# Autodesk Inventor assembly: linkage_system_test
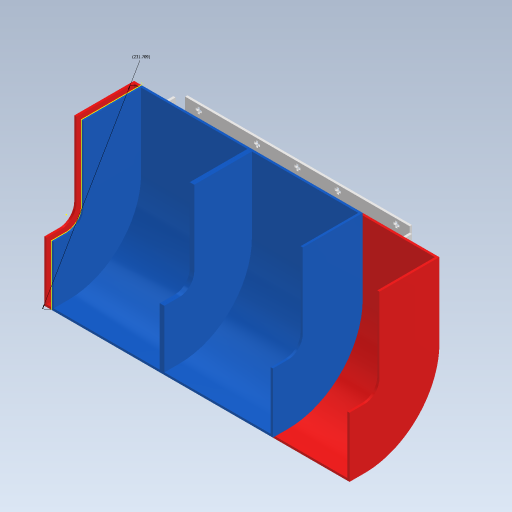
[picture p0: Inventor's stored thumbnail of the model, 512x512]
Saved by Autodesk Inventor 2023 (Build 270158000, 158)
## iProperties
Created: 2023-05-05
Part Number: linkage_system_test
Document SubType Name: Assembly
Designer: 陳詩穎
Author: 陳詩穎
## Documents named in this file (14)
- C:\Users\Johnny Jou\Documents\GitHub\Areo_Rider_Cabin\Expansion\test\linkage_system_test.iam
- C:\Users\Johnny Jou\Documents\GitHub\Areo_Rider_Cabin\Expansion\test\plate_expansion.ipt
- C:\Users\Johnny Jou\Documents\GitHub\Areo_Rider_Cabin\Expansion\test\零件1.ipt
- C:\Users\Johnny Jou\Documents\GitHub\Areo_Rider_Cabin\Expansion\test\adjustable.ipt
- C:\Users\Johnny Jou\Documents\GitHub\Areo_Rider_Cabin\Expansion\test\零件4.ipt
- C:\Users\Johnny Jou\Documents\GitHub\Areo_Rider_Cabin\Expansion\test\零件5.ipt
- C:\Users\Johnny Jou\Documents\GitHub\Areo_Rider_Cabin\Expansion\test\零件7.ipt
- C:\Users\Johnny Jou\Documents\GitHub\Areo_Rider_Cabin\Airfoil & Nuzzle\nuzzle\nuzzle_v2_0327.ipt
- C:\Users\Johnny Jou\Documents\GitHub\Areo_Rider_Cabin\Airfoil & Nuzzle\nuzzle\nuzzle_v2_0516.ipt
- C:\Users\Johnny Jou\Documents\GitHub\Areo_Rider_Cabin\Airfoil & Nuzzle\nuzzle\nuzzle_v2_0516_2.ipt
- C:\Users\Johnny Jou\Documents\GitHub\Areo_Rider_Cabin\Expansion\test\零件8.ipt
- C:\Users\Johnny Jou\Documents\GitHub\Areo_Rider_Cabin\Expansion\test\零件9.ipt
- C:\Users\Johnny Jou\Documents\GitHub\Areo_Rider_Cabin\Expansion\test\零件10.ipt
- C:\Users\Johnny Jou\Documents\GitHub\Areo_Rider_Cabin\Expansion\test\零件12.ipt
## Components (32 placed, 13 different names)
1. plate_expansion:1 — 貼合:1, 齊平:1, 貼合:2, 齊平:2, 齊平:6, 貼合:13, 齊平:8, 齊平:20
2. 零件1:1 — 齊平:2, 齊平:6, 貼合:13, 角度:1, 貼合:50, 貼合:112, 貼合:113, 貼合:126, 貼合:127
3. 零件1:2 — 貼合:1, 齊平:1, 貼合:2, 插入:10, 貼合:49, 貼合:51, 貼合:137, 貼合:138
4. adjustable:6 — 插入:10, 貼合:130, 貼合:131, 貼合:132, 貼合:133
5. 零件4:1 — 齊平:5, 貼合:18, 貼合:33, 貼合:100, 貼合:129, 貼合:140, 貼合:155, 貼合:170
6. 零件4:2 — 齊平:4, 齊平:5, 貼合:17, 貼合:18, 貼合:101, 貼合:115
7. 零件4:3 — 齊平:3, 齊平:4, 貼合:16, 齊平:11, 貼合:60
8. 零件4:4 — 齊平:3, 貼合:16, 貼合:17, 角度:1, 貼合:72
9. 零件5:1 — 齊平:8, 貼合:33, 齊平:11, 貼合:37, 貼合:38, 貼合:39, 貼合:40, 貼合:60, 貼合:72, 貼合:100, 貼合:101
10. nuzzle_v2_0327:1 — 貼合:43, 貼合:44, 齊平:20
11. 零件7:1 — 貼合:37, 貼合:38, 貼合:39, 齊平:14, 齊平:15, 貼合:90
12. 零件7:2 — 貼合:40, 齊平:14, 齊平:15, 貼合:91
13. nuzzle_v2_0516:1 — 貼合:43, 貼合:44, 貼合:45, 貼合:46, 貼合:89, 齊平:22
14. nuzzle_v2_0516_2:1 — 貼合:45, 貼合:46, 貼合:88, 齊平:21, 角度:2
15. 零件8:1 — 貼合:49, 貼合:50, 貼合:51
16. 零件9:1 — 貼合:88, 貼合:90, 齊平:21
17. 零件10:1 — 貼合:89, 貼合:91, 齊平:22
18. adjustable:18 — 貼合:112, 貼合:113, 貼合:133, 貼合:152
19. adjustable:19 — 貼合:115, 貼合:142, 貼合:157, 貼合:158
20. adjustable:23 — 貼合:126, 貼合:127, 貼合:139
21. adjustable:24 — 貼合:129, 貼合:140, 貼合:167, 貼合:168, 貼合:169
22. adjustable:28 — 貼合:130, 貼合:131, 貼合:132
23. adjustable:29 — 貼合:138, 貼合:139
24. adjustable:30 — 貼合:137
25. adjustable:31 — 貼合:142, 貼合:145, 貼合:146, 貼合:149, 貼合:150, 貼合:158, 貼合:159
26. adjustable:32 — 貼合:145, 貼合:146, 貼合:154
27. 零件12:2 — 貼合:149, 貼合:150, 貼合:159
28. 零件12:3 — 貼合:152, 貼合:154, 貼合:155, 貼合:157
29. adjustable:33 — 貼合:169
30. adjustable:34 — 貼合:166, 貼合:170
31. 零件12:4
32. 零件12:5 — 貼合:166, 貼合:167, 貼合:168
## Relationships (87: Mate 71, Flush 13, Angle 2, Insert 1)
- 貼合:1 [Mate]: plate_expansion:1 ↔ 零件1:2
- 齊平:1 [Flush]: plate_expansion:1 ↔ 零件1:2
- 貼合:2 [Mate]: plate_expansion:1 ↔ 零件1:2
- 齊平:2 [Flush]: plate_expansion:1 ↔ 零件1:1
- 插入:10 [Insert]: 零件1:2 ↔ adjustable:6
- 齊平:3 [Flush]: 零件4:3 ↔ 零件4:4
- 齊平:4 [Flush]: 零件4:2 ↔ 零件4:3
- 齊平:5 [Flush]: 零件4:1 ↔ 零件4:2
- 齊平:6 [Flush]: plate_expansion:1 ↔ 零件1:1
- 貼合:13 [Mate]: plate_expansion:1 ↔ 零件1:1
- 貼合:16 [Mate]: 零件4:3 ↔ 零件4:4
- 貼合:17 [Mate]: 零件4:2 ↔ 零件4:4
- 貼合:18 [Mate]: 零件4:1 ↔ 零件4:2
- 角度:1 [Angle] (180 deg): 零件1:1 ↔ 零件4:4
- 齊平:8 [Flush]: plate_expansion:1 ↔ 零件5:1
- 貼合:33 [Mate]: 零件4:1 ↔ 零件5:1
- 齊平:11 [Flush]: 零件4:3 ↔ 零件5:1
- 貼合:37 [Mate]: 零件5:1 ↔ 零件7:1
- 貼合:38 [Mate]: 零件5:1 ↔ 零件7:1
- 貼合:39 [Mate]: 零件5:1 ↔ 零件7:1
- 貼合:40 [Mate]: 零件5:1 ↔ 零件7:2
- 齊平:14 [Flush]: 零件7:1 ↔ 零件7:2
- 齊平:15 [Flush]: 零件7:1 ↔ 零件7:2
- 貼合:43 [Mate]: nuzzle_v2_0327:1 ↔ nuzzle_v2_0516:1
- 貼合:44 [Mate]: nuzzle_v2_0327:1 ↔ nuzzle_v2_0516:1
- 貼合:45 [Mate]: nuzzle_v2_0516:1 ↔ nuzzle_v2_0516_2:1
- 貼合:46 [Mate]: nuzzle_v2_0516:1 ↔ nuzzle_v2_0516_2:1
- 貼合:49 [Mate]: 零件1:2 ↔ 零件8:1
- 貼合:50 [Mate]: 零件1:1 ↔ 零件8:1
- 貼合:51 [Mate]: 零件1:2 ↔ 零件8:1
- 貼合:60 [Mate]: 零件4:3 ↔ 零件5:1
- 貼合:72 [Mate]: 零件4:4 ↔ 零件5:1
- 貼合:88 [Mate]: nuzzle_v2_0516_2:1 ↔ 零件9:1
- 貼合:89 [Mate]: nuzzle_v2_0516:1 ↔ 零件10:1
- 貼合:90 [Mate]: 零件7:1 ↔ 零件9:1
- 貼合:91 [Mate]: 零件7:2 ↔ 零件10:1
- 齊平:20 [Flush] (2 mm): plate_expansion:1 ↔ nuzzle_v2_0327:1
- 齊平:21 [Flush] (45 mm): nuzzle_v2_0516_2:1 ↔ 零件9:1
- 齊平:22 [Flush] (-44 mm): nuzzle_v2_0516:1 ↔ 零件10:1
- 貼合:100 [Mate]: 零件4:1 ↔ 零件5:1
- 貼合:101 [Mate]: 零件4:2 ↔ 零件5:1
- [Mate]: adjustable:18 ↔ adjustable:19
- [Mate]: adjustable:18 ↔ adjustable:19
- [Mate]: adjustable:18 ↔ adjustable:19
- 貼合:112 [Mate]: 零件1:1 ↔ adjustable:18
- 貼合:113 [Mate]: 零件1:1 ↔ adjustable:18
- 貼合:115 [Mate]: 零件4:2 ↔ adjustable:19
- [Mate]: adjustable:23 ↔ adjustable:24
- [Mate]: adjustable:23 ↔ adjustable:24
- [Mate]: adjustable:23 ↔ adjustable:24
- 貼合:126 [Mate]: 零件1:1 ↔ adjustable:23
- 貼合:127 [Mate]: 零件1:1 ↔ adjustable:23
- 貼合:129 [Mate]: 零件4:1 ↔ adjustable:24
- 貼合:130 [Mate]: adjustable:6 ↔ adjustable:28
- 貼合:131 [Mate]: adjustable:6 ↔ adjustable:28
- 貼合:132 [Mate]: adjustable:6 ↔ adjustable:28
- 貼合:133 [Mate]: adjustable:6 ↔ adjustable:18
- [Mate]: adjustable:29 ↔ adjustable:30
- [Mate]: adjustable:29 ↔ adjustable:30
- [Mate]: adjustable:29 ↔ adjustable:30
- 貼合:137 [Mate]: 零件1:2 ↔ adjustable:30
- 貼合:138 [Mate]: 零件1:2 ↔ adjustable:29
- 貼合:139 [Mate]: adjustable:23 ↔ adjustable:29
- 貼合:140 [Mate]: 零件4:1 ↔ adjustable:24
- 貼合:142 [Mate]: adjustable:19 ↔ adjustable:31
- 貼合:145 [Mate]: adjustable:31 ↔ adjustable:32
- 貼合:146 [Mate]: adjustable:31 ↔ adjustable:32
- 貼合:149 [Mate]: adjustable:31 ↔ 零件12:2
- 貼合:150 [Mate]: adjustable:31 ↔ 零件12:2
- 貼合:152 [Mate]: adjustable:18 ↔ 零件12:3
- 貼合:154 [Mate]: adjustable:32 ↔ 零件12:3
- 貼合:155 [Mate]: 零件4:1 ↔ 零件12:3
- 貼合:157 [Mate]: adjustable:19 ↔ 零件12:3
- 貼合:158 [Mate]: adjustable:19 ↔ adjustable:31
- 貼合:159 [Mate]: adjustable:31 ↔ 零件12:2
- [Mate]: adjustable:33 ↔ adjustable:34
- [Mate]: adjustable:33 ↔ adjustable:34
- [Mate]: adjustable:33 ↔ 零件12:4
- [Mate]: adjustable:33 ↔ 零件12:4
- [Mate]: adjustable:34 ↔ 零件12:5
- [Mate]: adjustable:33 ↔ 零件12:4
- 貼合:166 [Mate]: adjustable:34 ↔ 零件12:5
- 貼合:167 [Mate]: adjustable:24 ↔ 零件12:5
- 貼合:168 [Mate]: adjustable:24 ↔ 零件12:5
- 貼合:169 [Mate]: adjustable:24 ↔ adjustable:33
- 貼合:170 [Mate]: 零件4:1 ↔ adjustable:34
- 角度:2 [Angle] (0 deg): nuzzle_v2_0516_2:1
## Named parameters: d160_d98 = 0 mm, d161_d99 = 0 mm, d162_d100 = 0 mm, d174_d160_d98 = 0 mm, d175_d161_d99 = 0 mm, d176_d162_d100 = 0 mm, d192_d188 = 0 mm, d193_d189 = 0 mm, d194_d190 = 0 mm, d228_d222 = 0 mm, d229_d227 = 0 mm, d230_d210 = 0 mm, d231_d211 = 0 mm, d232_d214 = 0 mm, d233_d215 = 0 mm
